# Autodesk Inventor assembly: Assembly1
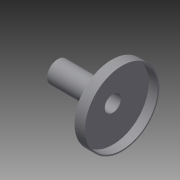
[picture p0: Inventor's stored thumbnail of the model, 180x180]
Saved by Autodesk Inventor 2013 (Build 170138000, 138)
## iProperties
Created: 2012-11-15
Part Number: Assembly1
Document SubType Name: Assembly
Designer: Breckenridge2 User
Author: Breckenridge2 User
## Documents named in this file (3)
- D:\Work_Suranga\3d_drawing_of_the_chamber\Educational_version\Assembly1.iam
- D:\Work_Suranga\3d_drawing_of_the_chamber\Educational_version\outer_ring_for_ground_shield.ipt
- D:\Work_Suranga\3d_drawing_of_the_chamber\Ground_shield_v2.ipt
## Components (2 placed, 2 different names)
1. Ground_shield_v2:1 — Insert:1
2. outer_ring_for_ground_shield:1 — Insert:1
## Relationships (1: Insert 1)
- Insert:1: Ground_shield_v2:1 ↔ outer_ring_for_ground_shield:1
